# Autodesk Inventor assembly: Montagem
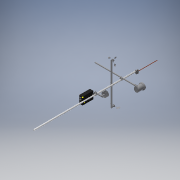
[picture p0: Inventor's stored thumbnail of the model, 180x180]
Saved by Autodesk Inventor 2019.4 (Build 234330000, 330)
## iProperties
Created: 2021-02-17
Part Number: Montagem
Material: Genérico
Document SubType Name: Assembly
Designer: Lattes
Author: Lattes
## Documents named in this file (20)
- C:\Users\Lattes\Documents\GitHub\estacao-meteorologica\Estrutura\estrutura_telhado\Montagem estação remota.iam
- C:\Users\Lattes\Documents\GitHub\estacao-meteorologica\Estrutura\estrutura_telhado\tubo_instrumentação_2500mm.ipt
- C:\Users\Lattes\Documents\GitHub\estacao-meteorologica\Estrutura\estrutura_telhado\fixador_haste_para_raio.ipt
- C:\Users\Lattes\Documents\GitHub\estacao-meteorologica\Estrutura\estrutura_telhado\haste_para_raio.ipt
- C:\Users\Lattes\Documents\GitHub\estacao-meteorologica\Estrutura\estrutura_telhado\parafuso u abraçadeira.ipt
- C:\Users\Lattes\Documents\GitHub\estacao-meteorologica\Estrutura\estrutura_telhado\fixador_externo_haste_para_raio.ipt
- C:\Users\Lattes\Documents\GitHub\estacao-meteorologica\Estrutura\estrutura_telhado\porca m6.ipt
- C:\Users\Lattes\Documents\GitHub\estacao-meteorologica\Estrutura\estrutura_telhado\suporte sensores 1m.ipt
- C:\Users\Lattes\Documents\GitHub\estacao-meteorologica\Estrutura\estrutura_telhado\Parafuso m3  30mm.ipt
- C:\Users\Lattes\Documents\GitHub\estacao-meteorologica\Estrutura\estrutura_telhado\fixador_suporte_sensor_solar.ipt
- C:\Users\Lattes\Documents\GitHub\estacao-meteorologica\Estrutura\estrutura_telhado\parafuso u abraçadeira menor.ipt
- C:\Users\Lattes\Documents\GitHub\estacao-meteorologica\Estrutura\estrutura_telhado\suporte sensores solares.ipt
- C:\Users\Lattes\Documents\GitHub\estacao-meteorologica\Estrutura\estrutura_telhado\parafuso-m6.ipt
- C:\Users\Lattes\Documents\GitHub\estacao-meteorologica\Estrutura\estrutura_telhado\ruela m6.ipt
- C:\Users\Lattes\Documents\GitHub\estacao-meteorologica\Estrutura\estrutura_telhado\caixa\caixa de instrumentação e controle.iam
- C:\Users\Lattes\Documents\GitHub\estacao-meteorologica\Estrutura\estrutura_telhado\anemometro.ipt
- C:\Users\Lattes\Documents\GitHub\estacao-meteorologica\Estrutura\estrutura_telhado\porca m3.ipt
- C:\Users\Lattes\Documents\GitHub\estacao-meteorologica\Estrutura\estrutura_telhado\wind_vane.ipt
- C:\Users\Lattes\Documents\GitHub\estacao-meteorologica\Estrutura\estrutura_telhado\Alojamento do Sensor de Temperatura e Umidade\alojamento sensor temperatura.iam
- C:\Users\Lattes\Documents\GitHub\estacao-meteorologica\Estrutura\estrutura_telhado\pluviometro.ipt
## Components (45 placed, 19 different names)
1. tubo_instrumentação_2500mm:1 — Inserir:1, Inserir:10, Inserir:15, Inserir:36, Inserir:40
2. fixador_haste_para_raio:2 — Inserir:1, Inserir:2, Inserir:3, Inserir:4
3. haste_para_raio:1 — Inserir:2
4. parafuso u abraçadeira:1 — Inserir:3
5. parafuso u abraçadeira:2 — Inserir:4, Inserir:5
6. fixador_externo_haste_para_raio:1 — Inserir:5, Inserir:6, Inserir:7, Inserir:8, Inserir:9
7. porca m6:1 — Inserir:8
8. porca m6:2 — Inserir:7
9. porca m6:3 — Inserir:9
10. porca m6:4 — Inserir:6
11. suporte sensores 1000 mm:1 — Inserir:10, Inserir:11, Inserir:12, Inserir:13, Inserir:14, Inserir:31, Inserir:32, Inserir:33, Inserir:34
12. parafuso u abraçadeira:3 — Inserir:11
13. porca m6:5 — Inserir:12
14. porca m6:6 — Inserir:13
15. Parafuso m3  30mm:1 — Inserir:14
16. fixador_suporte_sensor_solar:1 — Inserir:15, Inserir:16, Inserir:17, Inserir:18, Inserir:19, Inserir:20, Inserir:21, Inserir:22, Inserir:23, Inserir:24
17. parafuso u abraçadeira:6 — Inserir:37
18. parafuso u abraçadeira menor:1 — Inserir:16
19. parafuso u abraçadeira menor:2 — Inserir:17
20. porca m6:7 — Inserir:23
21. porca m6:8 — Inserir:21
22. porca m6:9 — Inserir:20
23. porca m6:10 — Inserir:22
24. porca m6:11 — Inserir:18
25. porca m6:12 — Inserir:19
26. suporte sensores solares:1 — Inserir:24, Inserir:25, Inserir:26, Inserir:41, Inserir:44, Inserir:45
27. parafuso-m6:1 — Inserir:28
28. parafuso-m6:2 — Inserir:27
29. ruela m6:1 — Inserir:26, Inserir:28
30. ruela m6:2 — Inserir:25, Inserir:27
31. porca m3:1 — Inserir:31
32. anemometro:1 — Inserir:33
33. wind_vane:1 — Inserir:32
34. porca m3:2 — Inserir:34
35. alojamento sensor temperatura:1 [sub-assembly] — Inserir:36, Inserir:37, Inserir:38, Inserir:39
36. porca m6:13 — Inserir:38
37. porca m6:14 — Inserir:39
38. caixa de instrumentação e controle:2 [sub-assembly] — Inserir:40
39. pluviometro:1 — Inserir:41, Inserir:42, Inserir:43
40. parafuso-m6:3 — Inserir:42
41. parafuso-m6:4 — Inserir:43
42. porca m6:15 — Inserir:46
43. porca m6:16 — Inserir:47
44. ruela m6:3 — Inserir:45, Inserir:47
45. ruela m6:4 — Inserir:44, Inserir:46
## Relationships (44: Insert 44)
- Inserir:1 (10 mm): tubo_instrumentação_2500mm:1 ↔ fixador_haste_para_raio:2
- Inserir:2: fixador_haste_para_raio:2 ↔ haste_para_raio:1
- Inserir:3 (-31 mm): fixador_haste_para_raio:2 ↔ parafuso u abraçadeira:1
- Inserir:4 (-31 mm): fixador_haste_para_raio:2 ↔ parafuso u abraçadeira:2
- Inserir:5 (-21 mm): parafuso u abraçadeira:2 ↔ fixador_externo_haste_para_raio:1
- Inserir:6: fixador_externo_haste_para_raio:1 ↔ porca m6:4
- Inserir:7: fixador_externo_haste_para_raio:1 ↔ porca m6:2
- Inserir:8: fixador_externo_haste_para_raio:1 ↔ porca m6:1
- Inserir:9: fixador_externo_haste_para_raio:1 ↔ porca m6:3
- Inserir:10: tubo_instrumentação_2500mm:1 ↔ suporte sensores 1000 mm:1
- Inserir:11 (-42.5 mm): suporte sensores 1000 mm:1 ↔ parafuso u abraçadeira:3
- Inserir:12: suporte sensores 1000 mm:1 ↔ porca m6:5
- Inserir:13: suporte sensores 1000 mm:1 ↔ porca m6:6
- Inserir:14: suporte sensores 1000 mm:1 ↔ Parafuso m3  30mm:1
- Inserir:15 (350 mm): tubo_instrumentação_2500mm:1 ↔ fixador_suporte_sensor_solar:1
- Inserir:16 (-10.5 mm): fixador_suporte_sensor_solar:1 ↔ parafuso u abraçadeira menor:1
- Inserir:17 (-10.5 mm): fixador_suporte_sensor_solar:1 ↔ parafuso u abraçadeira menor:2
- Inserir:18: fixador_suporte_sensor_solar:1 ↔ porca m6:11
- Inserir:19: fixador_suporte_sensor_solar:1 ↔ porca m6:12
- Inserir:20: fixador_suporte_sensor_solar:1 ↔ porca m6:9
- Inserir:21: fixador_suporte_sensor_solar:1 ↔ porca m6:8
- Inserir:22: fixador_suporte_sensor_solar:1 ↔ porca m6:10
- Inserir:23: fixador_suporte_sensor_solar:1 ↔ porca m6:7
- Inserir:24: fixador_suporte_sensor_solar:1 ↔ suporte sensores solares:1
- Inserir:25: suporte sensores solares:1 ↔ ruela m6:2
- Inserir:26: suporte sensores solares:1 ↔ ruela m6:1
- Inserir:27: parafuso-m6:2 ↔ ruela m6:2
- Inserir:28: parafuso-m6:1 ↔ ruela m6:1
- Inserir:31: suporte sensores 1000 mm:1 ↔ porca m3:1
- Inserir:32: suporte sensores 1000 mm:1 ↔ wind_vane:1
- Inserir:33: suporte sensores 1000 mm:1 ↔ anemometro:1
- Inserir:34: suporte sensores 1000 mm:1 ↔ porca m3:2
- Inserir:36: tubo_instrumentação_2500mm:1 ↔ alojamento sensor temperatura:1
- Inserir:37 (-43 mm): parafuso u abraçadeira:6 ↔ alojamento sensor temperatura:1
- Inserir:38: alojamento sensor temperatura:1 ↔ porca m6:13
- Inserir:39: alojamento sensor temperatura:1 ↔ porca m6:14
- Inserir:40: tubo_instrumentação_2500mm:1 ↔ caixa de instrumentação e controle:2
- Inserir:41: suporte sensores solares:1 ↔ pluviometro:1
- Inserir:42: pluviometro:1 ↔ parafuso-m6:3
- Inserir:43: pluviometro:1 ↔ parafuso-m6:4
- Inserir:44: suporte sensores solares:1 ↔ ruela m6:4
- Inserir:45: suporte sensores solares:1 ↔ ruela m6:3
- Inserir:46: porca m6:15 ↔ ruela m6:4
- Inserir:47: porca m6:16 ↔ ruela m6:3
